# Autodesk Inventor assembly: acrylic kinect bracket 2
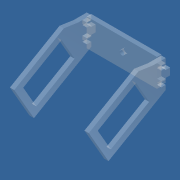
[picture p0: Inventor's stored thumbnail of the model, 180x180]
Saved by Autodesk Inventor 2012 (Build 160160000, 160)
## iProperties
Created: 2012-10-30
Part Number: acrylic kinect bracket 2
Document SubType Name: Assembly
Designer: Ed
Author: Ed
## Documents named in this file (3)
- C:\Users\Ed\Documents\masters\CAD\Kinect\acrylic kinect bracket 2.iam
- C:\Users\Ed\Documents\masters\CAD\Kinect\acrylic kinect bracket.ipt
- C:\Users\Ed\Documents\masters\CAD\Kinect\acrylic kinect plate.ipt
## Components (3 placed, 2 different names)
1. acrylic kinect bracket:1 — Flush:1, Flush:2, Mate:6, Mate:7, Mate:8
2. acrylic kinect bracket:2 — Flush:1, Flush:2, Mate:9
3. acrylic kinect plate:1 — Mate:6, Mate:7, Mate:8, Mate:9
## Relationships (6: Mate 4, Flush 2)
- Flush:1: acrylic kinect bracket:1 ↔ acrylic kinect bracket:2
- Flush:2: acrylic kinect bracket:1 ↔ acrylic kinect bracket:2
- Mate:6: acrylic kinect bracket:1 ↔ acrylic kinect plate:1
- Mate:7: acrylic kinect bracket:1 ↔ acrylic kinect plate:1
- Mate:8: acrylic kinect bracket:1 ↔ acrylic kinect plate:1
- Mate:9: acrylic kinect bracket:2 ↔ acrylic kinect plate:1
